# Autodesk Inventor assembly: ASY MSC 900.1 base frame
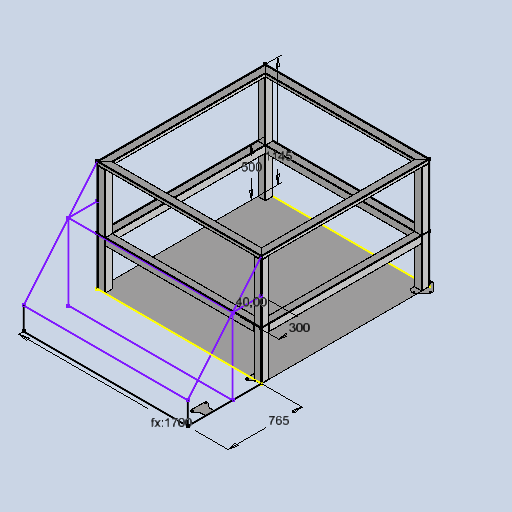
[picture p0: Inventor's stored thumbnail of the model, 512x512]
Saved by Autodesk Inventor 2025 (Build 290162010, 162A)
## iProperties
Created: 2024-05-19
Part Number: ASY MSC 900.1 base frame
Document SubType Name: Assembly
Designer: admin
Stock Number: ASY МОО 900.1 рама основания
_SolveAssemblyDoc: Frame Generator Solve Assembly
_Version: 15.0.0
Author: admin
## Documents named in this file (5)
- C:\Users\pokla\Documents\Inventor\Отстойник осветлитель\Manturovo_Se-clar-Gleb\Рама основания\ASY MSC 090 base frame.iam
- C:\Users\pokla\Documents\Inventor\Отстойник осветлитель\Manturovo_Se-clar-Gleb\MSC DIM 040 base frame.ipt
- C:\Users\pokla\Documents\Inventor\Отстойник осветлитель\Manturovo_Se-clar-Gleb\Рама основания\ASY МОО 040 рама основания\Frame\Frame 1716110745180.iam
- C:\Users\pokla\Documents\Inventor\Отстойник осветлитель\Manturovo_Se-clar-Gleb\MSC 127 flange frame heel.ipt
- C:\Users\pokla\Documents\Inventor\Отстойник осветлитель\Manturovo_Se-clar-Gleb\MSC 128 base plate.ipt
## Components (5 placed, 4 different names)
1. МОО DIM 040 рама основания.ipt:1
2. Frame 1716110745180.iam:1 [sub-assembly] — Rigid:3, Rigid:5
3. MSC 127 flange frame heel:3 — Rigid:3
4. MSC 128 base plate:1
5. MSC 128 base plate:2 — Rigid:5
## Relationships (2: WeldJoint 2)
- Rigid:3 [WeldJoint]: Frame 1716110745180.iam:1 ↔ MSC 127 flange frame heel:3
- Rigid:5 [WeldJoint]: Frame 1716110745180.iam:1 ↔ MSC 128 base plate:2
